# Autodesk Inventor assembly: rev1 base large wall
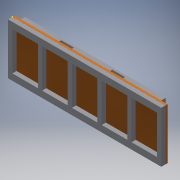
[picture p0: Inventor's stored thumbnail of the model, 180x180]
Saved by Autodesk Inventor 2017 (Build 210142000, 142)
## iProperties
Created: 2019-05-04
Part Number: rev1 base large wall
Document SubType Name: Assembly
Designer: Roman
Author: Roman
## Documents named in this file (7)
- C:\Users\Roman\Documents\CAD\enclosure rev1\rev2 base\rev1 large wall\rev1 base large wall.iam
- C:\Users\Roman\Documents\CAD\enclosure rev1\rev2 base\rev1 large wall\rev1 base large wall backplane.ipt
- C:\Users\Roman\Documents\CAD\enclosure rev1\rev2 base\rev1 large wall\rev1 base large wall h stud.ipt
- C:\Users\Roman\Documents\CAD\enclosure rev1\rev2 base\rev1 large wall\rev1 base large wall v stud.ipt
- C:\Users\Roman\Documents\CAD\enclosure rev1\rev2 base\rev1 tube.ipt
- C:\Users\Roman\Documents\CAD\enclosure rev1\rev2 base\rev1 large wall\rev1 base large wall plank middle.ipt
- C:\Users\Roman\Documents\CAD\enclosure rev1\rev2 base\rev1 large wall\rev1 base large wall plank side.ipt
## Components (20 placed, 6 different names)
1. rev1 base large wall backplane:1 — Mate:1, Mate:2, Flush:1, Flush:2, Flush:3, Flush:4, Mate:4, Flush:5, Mate:5, Flush:6, Mate:6, Flush:7, Flush:8, Flush:9, Mate:8, Mate:11, Mate:12, Flush:11, Flush:12
2. rev1 base large wall h stud:1 — Mate:1, Flush:1, Flush:2, Mate:3
3. rev1 base large wall h stud:2 — Mate:2, Flush:3, Flush:4
4. rev1 tube:1 — Mate:5, Flush:6, Flush:8, Mate:10
5. rev1 tube:2 — Mate:6, Flush:7, Flush:9, Mate:7, Flush:10, Mate:9
6. rev1 base large wall plank middle:1 — Mate:7, Mate:8, Flush:10
7. rev1 base large wall plank side:1 — Mate:9, Mate:12, Flush:11
8. rev1 base large wall plank side:2 — Mate:10, Mate:11, Flush:12
9. rev1 base large wall v stud:1 — Mate:3, Mate:4, Flush:5
10. rev1 base large wall v stud:2
11. rev1 base large wall v stud:3
12. rev1 base large wall v stud:4
13. rev1 base large wall v stud:5
14. rev1 base large wall v stud:6
15. rev1 base large wall v stud:7
16. rev1 base large wall v stud:8
17. rev1 base large wall v stud:9
18. rev1 base large wall v stud:10
19. rev1 base large wall v stud:11
20. rev1 base large wall v stud:12
## Component patterns: (12 elements, first: rev1 base large wall v stud:1)
## Relationships (24: Mate 12, Flush 12)
- Mate:1: rev1 base large wall backplane:1 ↔ rev1 base large wall h stud:1
- Mate:2: rev1 base large wall backplane:1 ↔ rev1 base large wall h stud:2
- Flush:1: rev1 base large wall backplane:1 ↔ rev1 base large wall h stud:1
- Flush:2: rev1 base large wall backplane:1 ↔ rev1 base large wall h stud:1
- Flush:3: rev1 base large wall backplane:1 ↔ rev1 base large wall h stud:2
- Flush:4: rev1 base large wall backplane:1 ↔ rev1 base large wall h stud:2
- Mate:3: rev1 base large wall h stud:1 ↔ rev1 base large wall v stud:1
- Mate:4: rev1 base large wall backplane:1 ↔ rev1 base large wall v stud:1
- Flush:5: rev1 base large wall backplane:1 ↔ rev1 base large wall v stud:1
- Mate:5: rev1 base large wall backplane:1 ↔ rev1 tube:1
- Flush:6: rev1 base large wall backplane:1 ↔ rev1 tube:1
- Mate:6: rev1 base large wall backplane:1 ↔ rev1 tube:2
- Flush:7: rev1 base large wall backplane:1 ↔ rev1 tube:2
- Flush:8 (508 mm): rev1 base large wall backplane:1 ↔ rev1 tube:1
- Flush:9 (508 mm): rev1 base large wall backplane:1 ↔ rev1 tube:2
- Mate:7: rev1 tube:2 ↔ rev1 base large wall plank middle:1
- Mate:8: rev1 base large wall backplane:1 ↔ rev1 base large wall plank middle:1
- Flush:10: rev1 tube:2 ↔ rev1 base large wall plank middle:1
- Mate:9: rev1 tube:2 ↔ rev1 base large wall plank side:1
- Mate:10: rev1 tube:1 ↔ rev1 base large wall plank side:2
- Mate:11: rev1 base large wall backplane:1 ↔ rev1 base large wall plank side:2
- Mate:12: rev1 base large wall backplane:1 ↔ rev1 base large wall plank side:1
- Flush:11: rev1 base large wall backplane:1 ↔ rev1 base large wall plank side:1
- Flush:12: rev1 base large wall backplane:1 ↔ rev1 base large wall plank side:2
